# Autodesk Inventor assembly: tempAsm
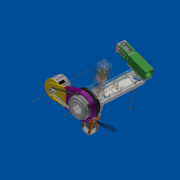
[picture p0: Inventor's stored thumbnail of the model, 180x180]
Saved by Autodesk Inventor 2018 (Build 220112000, 112)
## iProperties
Created: 2020-03-07
Part Number: tempAsm
Document SubType Name: Assembly
Designer: Bunny320
Author: Bunny320
## Documents named in this file (9)
- C:\Users\Bunny320\Desktop\sechs\4-CAD\tempAsm.iam
- C:\Users\Bunny320\Desktop\sechs\4-CAD\10-J1.iam
- C:\Users\Bunny320\Desktop\sechs\4-CAD\20-J2.iam
- C:\Users\Bunny320\Desktop\sechs\4-CAD\30-J3.iam
- C:\Users\Bunny320\Documents\Inventor\Content Center Files\R2018\en-US\ISO 4762(1)\DIN EN ISO 4762 - M3 x 12.ipt
- C:\Users\Bunny320\Documents\Inventor\Content Center Files\R2018\en-US\ISO 4762(1)\DIN EN ISO 4762 - M3 x 20.ipt
- C:\Users\Bunny320\Documents\Inventor\Content Center Files\R2018\en-US\DIN EN ISO 4032\DIN EN ISO 4032 - M3.ipt
- C:\Users\Bunny320\Documents\Inventor\Content Center Files\R2018\en-US\ISO 4762(1)\DIN EN ISO 4762 - M3 x 25.ipt
- C:\Users\Bunny320\Desktop\sechs\4-CAD\40-J4.iam
## Components (22 placed, 8 different names)
1. 10-J1:1 [sub-assembly] — Flush:1, Flush:2, Flush:3, Mate:1, Mate:2, Mate:3, Mate:4, Mate:5, Mate:6, Mate:9, Mate:13, Mate:15, Mate:17, Mate:19, Mate:25, Mate:27, Mate:29
2. 20-J2:1 [sub-assembly] — Mate:1, Mate:2, Mate:3, Flush:4, Mate:10, Mate:14, Mate:16, Mate:18, Mate:20, Mate:26, Mate:28, Mate:30, Mate:33, Mate:34, Mate:36, Mate:39, Mate:41, Mate:43, Mate:45, Mate:47, Mate:49
3. 30-J3:1 [sub-assembly] — Mate:4, Mate:5, Mate:6, Flush:4, Mate:31, Mate:32, Mate:38, Mate:40, Mate:42, Mate:44, Mate:46, Mate:48, Mate:50, Mate:51, Mate:52
4. DIN EN ISO 4762 M3 x 12:1 — Mate:9, Mate:10
5. DIN EN ISO 4762 M3 x 12:3 — Mate:13, Mate:14
6. DIN EN ISO 4762 M3 x 12:4 — Mate:15, Mate:16
7. DIN EN ISO 4762 M3 x 12:5 — Mate:17, Mate:18
8. DIN EN ISO 4762 M3 x 12:6 — Mate:19, Mate:20
9. DIN EN ISO 4762 M3 x 12:9 — Mate:25, Mate:26
10. DIN EN ISO 4762 M3 x 12:10 — Mate:27, Mate:28
11. DIN EN ISO 4762 M3 x 12:11 — Mate:29, Mate:30
12. DIN EN ISO 4762 M3 x 20:1 — Mate:31, Mate:32, Mate:35
13. DIN EN ISO 4762 M3 x 20:2 — Mate:33, Mate:34, Mate:37
14. DIN EN ISO 4032 M3:1 — Mate:35, Mate:36
15. DIN EN ISO 4032 M3:2 — Mate:37, Mate:38
16. DIN EN ISO 4762 M3 x 25:1 — Mate:39, Mate:40
17. DIN EN ISO 4762 M3 x 25:2 — Mate:41, Mate:42
18. DIN EN ISO 4762 M3 x 25:3 — Mate:43, Mate:44
19. DIN EN ISO 4762 M3 x 25:4 — Mate:45, Mate:46
20. DIN EN ISO 4762 M3 x 25:5 — Mate:47, Mate:48
21. DIN EN ISO 4762 M3 x 25:6 — Mate:49, Mate:50
22. 40-J4:1 [sub-assembly] — Mate:51, Mate:52
## Relationships (48: Mate 44, Flush 4)
- Flush:1: 10-J1:1
- Flush:2: 10-J1:1
- Flush:3: 10-J1:1
- Mate:1: 10-J1:1 ↔ 20-J2:1
- Mate:2: 10-J1:1 ↔ 20-J2:1
- Mate:3: 10-J1:1 ↔ 20-J2:1
- Mate:4: 10-J1:1 ↔ 30-J3:1
- Mate:5: 10-J1:1 ↔ 30-J3:1
- Mate:6: 10-J1:1 ↔ 30-J3:1
- Flush:4: 20-J2:1 ↔ 30-J3:1
- Mate:9: 10-J1:1 ↔ DIN EN ISO 4762 M3 x 12:1
- Mate:10: 20-J2:1 ↔ DIN EN ISO 4762 M3 x 12:1
- Mate:13: 10-J1:1 ↔ DIN EN ISO 4762 M3 x 12:3
- Mate:14: 20-J2:1 ↔ DIN EN ISO 4762 M3 x 12:3
- Mate:15: 10-J1:1 ↔ DIN EN ISO 4762 M3 x 12:4
- Mate:16: 20-J2:1 ↔ DIN EN ISO 4762 M3 x 12:4
- Mate:17: 10-J1:1 ↔ DIN EN ISO 4762 M3 x 12:5
- Mate:18: 20-J2:1 ↔ DIN EN ISO 4762 M3 x 12:5
- Mate:19: 10-J1:1 ↔ DIN EN ISO 4762 M3 x 12:6
- Mate:20: 20-J2:1 ↔ DIN EN ISO 4762 M3 x 12:6
- Mate:25: 10-J1:1 ↔ DIN EN ISO 4762 M3 x 12:9
- Mate:26: 20-J2:1 ↔ DIN EN ISO 4762 M3 x 12:9
- Mate:27: 10-J1:1 ↔ DIN EN ISO 4762 M3 x 12:10
- Mate:28: 20-J2:1 ↔ DIN EN ISO 4762 M3 x 12:10
- Mate:29: 10-J1:1 ↔ DIN EN ISO 4762 M3 x 12:11
- Mate:30: 20-J2:1 ↔ DIN EN ISO 4762 M3 x 12:11
- Mate:31: 30-J3:1 ↔ DIN EN ISO 4762 M3 x 20:1
- Mate:32: 30-J3:1 ↔ DIN EN ISO 4762 M3 x 20:1
- Mate:33: 20-J2:1 ↔ DIN EN ISO 4762 M3 x 20:2
- Mate:34: 20-J2:1 ↔ DIN EN ISO 4762 M3 x 20:2
- Mate:35: DIN EN ISO 4762 M3 x 20:1 ↔ DIN EN ISO 4032 M3:1
- Mate:36: 20-J2:1 ↔ DIN EN ISO 4032 M3:1
- Mate:37: DIN EN ISO 4762 M3 x 20:2 ↔ DIN EN ISO 4032 M3:2
- Mate:38: 30-J3:1 ↔ DIN EN ISO 4032 M3:2
- Mate:39: 20-J2:1 ↔ DIN EN ISO 4762 M3 x 25:1
- Mate:40: 30-J3:1 ↔ DIN EN ISO 4762 M3 x 25:1
- Mate:41: 20-J2:1 ↔ DIN EN ISO 4762 M3 x 25:2
- Mate:42: 30-J3:1 ↔ DIN EN ISO 4762 M3 x 25:2
- Mate:43: 20-J2:1 ↔ DIN EN ISO 4762 M3 x 25:3
- Mate:44: 30-J3:1 ↔ DIN EN ISO 4762 M3 x 25:3
- Mate:45: 20-J2:1 ↔ DIN EN ISO 4762 M3 x 25:4
- Mate:46: 30-J3:1 ↔ DIN EN ISO 4762 M3 x 25:4
- Mate:47: 20-J2:1 ↔ DIN EN ISO 4762 M3 x 25:5
- Mate:48: 30-J3:1 ↔ DIN EN ISO 4762 M3 x 25:5
- Mate:49: 20-J2:1 ↔ DIN EN ISO 4762 M3 x 25:6
- Mate:50: 30-J3:1 ↔ DIN EN ISO 4762 M3 x 25:6
- Mate:51: 30-J3:1 ↔ 40-J4:1
- Mate:52: 30-J3:1 ↔ 40-J4:1
